# Autodesk Inventor assembly: Cylinder Tube
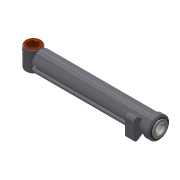
[picture p0: Inventor's stored thumbnail of the model, 180x180]
Saved by Autodesk Inventor 2022 Beta2 (Build 260130000, 130) ContinuousBuild 0
## iProperties
Created: 2002-06-13
Part Number: Cylinder Tube
Document SubType Name: Assembly
Designer: Joe M
Engineer: Joe M
Control State: 0
Master: False
Checked Out: False
Shininess: 64.0
Length Units: 11269
Angle Units: 11279
Time Units: 11290
Mass Units: 11283
Length Display Precision: 3
Angle Display Precision: 2
Density: 0.0
Volumn: 0.0
Area: 0.0
PropertySet Name: Model Information
Author: Joe M
## Documents named in this file (7)
- C:\Autodesk Inventor 2021 Intro Practice Files\BOM\Cylinder Tube.iam
- C:\Autodesk Inventor 2021 Intro Practice Files\BOM\3136 1144 59.ipt
- C:\Autodesk Inventor 2021 Intro Practice Files\BOM\3136 7048 80.ipt
- C:\Autodesk Inventor 2021 Intro Practice Files\BOM\0544 1100 09.ipt
- C:\Autodesk Inventor 2021 Intro Practice Files\BOM\3136 7009 55.ipt
- C:\Autodesk Inventor 2021 Intro Practice Files\BOM\3136 7009 59.ipt
- C:\Autodesk Inventor 2021 Intro Practice Files\BOM\3136 1074 64.ipt
## Components (7 placed, 6 different names)
1. 3136 1144 59:1 — Insert:2, Insert:3, Mate:1, Mate:2, Insert:1
2. 3136 7048 80:1 — Insert:2
3. 3136 7048 80:2 — Insert:3
4. 0544 1100 09:1 — Mate:1, Mate:2
5. 3136 7009 55:1 — Mate:3, Mate:4
6. 3136 7009 59:1 — Mate:5, Mate:6, Insert:1
7. 3136 1074 64:1 — Mate:3, Mate:4, Mate:5, Mate:6
## Relationships (9: Mate 6, Insert 3)
- Insert:2: 3136 1144 59:1 ↔ 3136 7048 80:1
- Insert:3: 3136 1144 59:1 ↔ 3136 7048 80:2
- Mate:1: 3136 1144 59:1 ↔ 0544 1100 09:1
- Mate:2 (30 mm): 3136 1144 59:1 ↔ 0544 1100 09:1
- Mate:3: 3136 7009 55:1 ↔ 3136 1074 64:1
- Mate:4: 3136 7009 55:1 ↔ 3136 1074 64:1
- Mate:5: 3136 7009 59:1 ↔ 3136 1074 64:1
- Mate:6 (0.075 mm): 3136 7009 59:1 ↔ 3136 1074 64:1
- Insert:1: 3136 1144 59:1 ↔ 3136 7009 59:1
## Named parameters: d0_d2 = 0 mm, d1_d7 = 0 mm, d2_d10 = 0 mm, d3_d11 = 30 mm
